# Autodesk Inventor assembly: TailAssembly
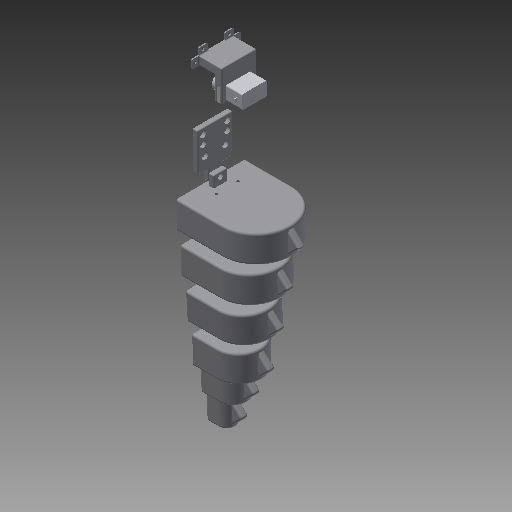
[picture p0: Inventor's stored thumbnail of the model, 512x512]
Saved by Autodesk Inventor 2018 (Build 220112000, 112)
## iProperties
Created: 2017-11-24
Part Number: TailAssembly
Document SubType Name: Assembly
Designer: reide
Author: reide
## Documents named in this file (8)
- C:\Users\reide\OneDrive\Documents\Inventor\TSA\2018\Animatronics\Tortoise\Tail\TailAssembly.iam
- C:\Users\reide\OneDrive\Documents\Inventor\TSA\2018\Animatronics\Tortoise\Tail\Tail_Servo_Mount.ipt
- C:\Users\reide\OneDrive\Documents\Inventor\TSA\2018\Animatronics\Tortoise\Tail\Tail_Mount.ipt
- C:\Users\reide\OneDrive\Documents\Inventor\TSA\2018\Animatronics\Tortoise\Tail\Tail4.ipt
- C:\Users\reide\OneDrive\Documents\Inventor\TSA\2018\Animatronics\Tortoise\Tail\Tail5.ipt
- C:\Users\reide\OneDrive\Documents\Inventor\TSA\2018\Animatronics\Tortoise\Tail\Tail6.ipt
- C:\Users\reide\OneDrive\Documents\Inventor\TSA\2018\Animatronics\Tortoise\Tail\Tail3.ipt
- C:\Users\reide\OneDrive\Documents\Inventor\TSA\2018\Animatronics\Tortoise\Mock Parts\servo (2).ipt
## Components (7 placed, 7 different names)
1. Tail_Servo_Mount:1 — Flush:1, Flush:3, Mate:8, Mate:9
2. Tail_Mount:1 — Flush:1, Mate:5, Mate:6
3. Tail4:1 — Mate:1, Mate:3, Mate:5, Flush:2, Mate:7
4. Tail5:1 — Mate:1, Mate:2, Mate:3, Mate:4
5. Tail6:1 — Mate:2, Mate:4
6. Tail3:1 — Mate:6, Flush:2, Mate:7
7. servo (2):1 — Flush:3, Mate:8, Mate:9
## Relationships (12: Mate 9, Flush 3)
- Flush:1: Tail_Servo_Mount:1 ↔ Tail_Mount:1
- Mate:1: Tail4:1 ↔ Tail5:1
- Mate:2: Tail5:1 ↔ Tail6:1
- Mate:3: Tail4:1 ↔ Tail5:1
- Mate:4: Tail5:1 ↔ Tail6:1
- Mate:5: Tail_Mount:1 ↔ Tail4:1
- Mate:6: Tail_Mount:1 ↔ Tail3:1
- Flush:2: Tail4:1 ↔ Tail3:1
- Mate:7: Tail4:1 ↔ Tail3:1
- Flush:3: Tail_Servo_Mount:1 ↔ servo (2):1
- Mate:8: Tail_Servo_Mount:1 ↔ servo (2):1
- Mate:9: Tail_Servo_Mount:1 ↔ servo (2):1
